# Autodesk Inventor assembly: upper_arm_1
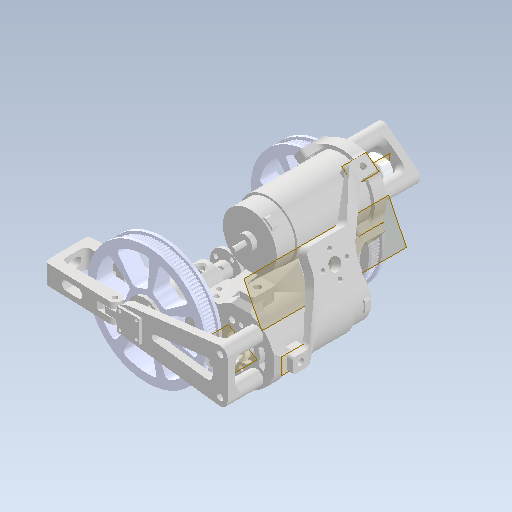
[picture p0: Inventor's stored thumbnail of the model, 512x512]
Saved by Autodesk Inventor 2020 (Build 240168000, 168)
## iProperties
Created: 2019-10-15
Part Number: upper_arm_1
Document SubType Name: Assembly
Designer: psrob
Author: psrob
## Documents named in this file (5)
- E:\projects-2\haptic device gen3\hardware\upper_arm_1.iam
- E:\projects-2\haptic device gen3\hardware\belt_reducer_1.iam
- E:\projects-2\haptic device gen3\hardware\arm_frame_1.ipt
- E:\projects-2\haptic device gen3\hardware\arm_frame_2.ipt
- E:\projects-2\haptic device gen3\hardware\arm_frame_3.ipt
## Components (5 placed, 4 different names)
1. belt_reducer_1:1 [sub-assembly] — Insert:1, Tangent:1, Flush:1, Insert:3, Flush:3, Insert:4, Flush:7
2. belt_reducer_1:2 [sub-assembly] — Insert:1, Tangent:1, Flush:2, Insert:2, Flush:4, Insert:5, Flush:8
3. arm_frame_1:1 — Flush:1, Flush:2, Insert:2, Insert:3
4. arm_frame_2:1 — Flush:3, Flush:4, Insert:4, Insert:5, Flush:5
5. arm_frame_3:1 — Flush:6, Flush:7, Flush:8
## Relationships (14: Flush 8, Insert 5, Tangent 1)
- Insert:1 (10 mm): belt_reducer_1:1 ↔ belt_reducer_1:2
- Tangent:1 (5 mm): belt_reducer_1:1 ↔ belt_reducer_1:2
- Flush:1: belt_reducer_1:1 ↔ arm_frame_1:1
- Flush:2: belt_reducer_1:2 ↔ arm_frame_1:1
- Insert:2: belt_reducer_1:2 ↔ arm_frame_1:1
- Insert:3: belt_reducer_1:1 ↔ arm_frame_1:1
- Flush:3: belt_reducer_1:1 ↔ arm_frame_2:1
- Flush:4: belt_reducer_1:2 ↔ arm_frame_2:1
- Insert:4: belt_reducer_1:1 ↔ arm_frame_2:1
- Insert:5: belt_reducer_1:2 ↔ arm_frame_2:1
- Flush:5: arm_frame_2:1
- Flush:6: arm_frame_3:1
- Flush:7: belt_reducer_1:1 ↔ arm_frame_3:1
- Flush:8: belt_reducer_1:2 ↔ arm_frame_3:1
